# Autodesk Inventor assembly: Assembly1
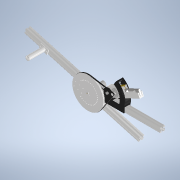
[picture p0: Inventor's stored thumbnail of the model, 180x180]
Saved by Autodesk Inventor 2022 (Build 260153000, 153)
## iProperties
Created: 2022-01-28
Part Number: Assembly1
Document SubType Name: Assembly
Designer: Martijn
Author: Martijn
## Documents named in this file (23)
- D:\phd\git\1dofsetup\Assembly1.iam
- D:\phd\git\1dofsetup\30x30x50.ipt
- D:\phd\git\1dofsetup\bearing_mount.ipt
- D:\phd\git\1dofsetup\force_measurement_thingy.ipt
- D:\phd\git\1dofsetup\NEMA 17.ipt
- D:\phd\git\1dofsetup\pololu-universal-aluminum-mounting-hub-for-5mm-shaft-m3-holes.ipt
- D:\phd\git\1dofsetup\space_plate.ipt
- D:\phd\git\1dofsetup\pololu-universal-aluminum-mounting-hub-for-8mm-shaft-m3-holes.ipt
- D:\phd\git\1dofsetup\SKF_608-2ZZ.ipt
- D:\phd\git\1dofsetup\just_pulley.ipt
- D:\phd\git\1dofsetup\GT2_16T.ipt
- D:\phd\git\1dofsetup\force_measurement_plate.ipt
- D:\phd\git\1dofsetup\load_cell.ipt
- D:\phd\git\1dofsetup\fixation_circle.ipt
- D:\phd\git\1dofsetup\fixation_plate2.ipt
- D:\phd\git\1dofsetup\8mm_to 6.35mm_kaplin.ipt
- D:\phd\git\1dofsetup\axis1.ipt
- D:\phd\git\1dofsetup\Lock Collar 8mm.ipt
- D:\phd\git\1dofsetup\belt.ipt
- D:\phd\git\1dofsetup\handle.ipt
- D:\phd\git\1dofsetup\bearing_mount3.ipt
- D:\phd\git\1dofsetup\axis2.ipt
- D:\phd\git\1dofsetup\load_cell_mounting_block2.ipt
## Components (27 placed, 22 different names)
1. 30x30x50:1 — Mate:96, Flush:34, Mate:106, Flush:35, Flush:36, Mate:118, Flush:38, Mate:131, Flush:44, Mate:132, Mate:133
2. 30x30x50:2 — Mate:29, Flush:10, Mate:107, Mate:108, Flush:37, Flush:39, Mate:120, Flush:40
3. force_measurement_thingy:1 — Mate:99, Mate:100, Mate:101, Mate:102, Mate:103, Mate:104, Mate:135, Angle:1
4. NEMA 17:1 — Mate:6, Mate:102, Mate:103, Mate:104, Mate:105, Mate:112
5. pololu-universal-aluminum-mounting-hub-for-5mm-shaft-m3-holes:1 — Mate:6, Mate:35, Mate:37
6. space_plate:1 — Flush:39, Mate:120, Flush:40, Mate:124, Flush:41, Flush:42
7. pololu-universal-aluminum-mounting-hub-for-8mm-shaft-m3-holes:1 — Mate:115, Mate:116, Mate:117, Mate:123, Flush:43
8. SKF_608-2ZZ:2 — Mate:136
9. just_pulley:1 — Mate:106, Flush:35, Mate:109, Mate:110, Mate:111, Mate:113, Mate:115, Mate:116, Mate:117, Flush:36, Mate:127, Mate:128, Mate:130
10. SKF_608-2ZZ:4 — Mate:110, Mate:127
11. GT2_16T:1 — Mate:36, Mate:105, Mate:114
12. force_measurement_plate:2 — Mate:29, Flush:10, Mate:78, Mate:100, Mate:134, Mate:137, Mate:138
13. load_cell:1 — Mate:101, Mate:135, Angle:1, Mate:139
14. fixation_circle:1 — Mate:35, Mate:36, Mate:37
15. fixation_plate2:1 — Mate:118, Flush:38, Mate:122, Mate:125, Mate:126, Mate:133
16. 8mm_to 6.35mm_kaplin:1 — Mate:122, Mate:129
17. bearing_mount:1 — Mate:107, Mate:108, Mate:109, Mate:111, Flush:37
18. axis1:1 — Mate:75, Mate:77, Flush:30, Mate:99, Mate:136
19. Lock Collar 8mm:1 — Mate:75
20. Lock Collar 8mm:2 — Mate:77, Mate:78, Flush:30, Mate:134
21. belt:1 — Mate:112, Mate:113, Mate:114, Mate:130
22. handle:1 — Mate:96, Flush:34, Mate:123
23. bearing_mount3:1 — Mate:124, Flush:41, Flush:42, Mate:129
24. SKF_608-2ZZ:5 — Mate:125, Mate:126
25. axis2:1 — Mate:128, Flush:43, Mate:140
26. 30x30x50:3 — Mate:131, Flush:44, Mate:132
27. load_cell_mounting_block2:1 — Mate:137, Mate:138, Mate:139
## Relationships (63: Mate 49, Flush 13, Angle 1)
- Mate:6 (1 mm): NEMA 17:1 ↔ pololu-universal-aluminum-mounting-hub-for-5mm-shaft-m3-holes:1
- Mate:29: 30x30x50:2 ↔ force_measurement_plate:2
- Flush:10: 30x30x50:2 ↔ force_measurement_plate:2
- Mate:35: pololu-universal-aluminum-mounting-hub-for-5mm-shaft-m3-holes:1 ↔ fixation_circle:1
- Mate:36: GT2_16T:1 ↔ fixation_circle:1
- Mate:37: pololu-universal-aluminum-mounting-hub-for-5mm-shaft-m3-holes:1 ↔ fixation_circle:1
- Mate:75: axis1:1 ↔ Lock Collar 8mm:1
- Mate:77: axis1:1 ↔ Lock Collar 8mm:2
- Mate:78: force_measurement_plate:2 ↔ Lock Collar 8mm:2
- Flush:30 (0.5 mm): axis1:1 ↔ Lock Collar 8mm:2
- Mate:96: 30x30x50:1 ↔ handle:1
- Flush:34: 30x30x50:1 ↔ handle:1
- Mate:99: force_measurement_thingy:1 ↔ axis1:1
- Mate:100 (0.5 mm): force_measurement_thingy:1 ↔ force_measurement_plate:2
- Mate:101: force_measurement_thingy:1 ↔ load_cell:1
- Mate:102: force_measurement_thingy:1 ↔ NEMA 17:1
- Mate:103: force_measurement_thingy:1 ↔ NEMA 17:1
- Mate:104: force_measurement_thingy:1 ↔ NEMA 17:1
- Mate:105: NEMA 17:1 ↔ GT2_16T:1
- Mate:106: 30x30x50:1 ↔ just_pulley:1
- Flush:35: 30x30x50:1 ↔ just_pulley:1
- Mate:107: 30x30x50:2 ↔ bearing_mount:1
- Mate:108 (-50 mm): 30x30x50:2 ↔ bearing_mount:1
- Mate:109: just_pulley:1 ↔ bearing_mount:1
- Mate:110: just_pulley:1 ↔ SKF_608-2ZZ:4
- Mate:111: just_pulley:1 ↔ bearing_mount:1
- Mate:112: NEMA 17:1 ↔ belt:1
- Mate:113: just_pulley:1 ↔ belt:1
- Mate:114 (0.5 mm): GT2_16T:1 ↔ belt:1
- Mate:115: pololu-universal-aluminum-mounting-hub-for-8mm-shaft-m3-holes:1 ↔ just_pulley:1
- Mate:116: pololu-universal-aluminum-mounting-hub-for-8mm-shaft-m3-holes:1 ↔ just_pulley:1
- Mate:117: pololu-universal-aluminum-mounting-hub-for-8mm-shaft-m3-holes:1 ↔ just_pulley:1
- Flush:36: 30x30x50:1 ↔ just_pulley:1
- Flush:37: 30x30x50:2 ↔ bearing_mount:1
- Mate:118: 30x30x50:1 ↔ fixation_plate2:1
- Flush:38: 30x30x50:1 ↔ fixation_plate2:1
- Flush:39: 30x30x50:2 ↔ space_plate:1
- Mate:120: 30x30x50:2 ↔ space_plate:1
- Flush:40: 30x30x50:2 ↔ space_plate:1
- Mate:122: fixation_plate2:1 ↔ 8mm_to 6.35mm_kaplin:1
- Mate:123 (300 mm): pololu-universal-aluminum-mounting-hub-for-8mm-shaft-m3-holes:1 ↔ handle:1
- Mate:124: space_plate:1 ↔ bearing_mount3:1
- Flush:41: space_plate:1 ↔ bearing_mount3:1
- Flush:42: space_plate:1 ↔ bearing_mount3:1
- Mate:125: fixation_plate2:1 ↔ SKF_608-2ZZ:5
- Mate:126: fixation_plate2:1 ↔ SKF_608-2ZZ:5
- Mate:127 (0.5 mm): just_pulley:1 ↔ SKF_608-2ZZ:4
- Mate:128: just_pulley:1 ↔ axis2:1
- Flush:43: pololu-universal-aluminum-mounting-hub-for-8mm-shaft-m3-holes:1 ↔ axis2:1
- Mate:129 (5 mm): 8mm_to 6.35mm_kaplin:1 ↔ bearing_mount3:1
- Mate:130 (0.5 mm): just_pulley:1 ↔ belt:1
- Mate:131: 30x30x50:1 ↔ 30x30x50:3
- Flush:44: 30x30x50:1 ↔ 30x30x50:3
- Mate:132 (-60 mm): 30x30x50:1 ↔ 30x30x50:3
- Mate:133 (-60 mm): 30x30x50:1 ↔ fixation_plate2:1
- Mate:134: force_measurement_plate:2 ↔ Lock Collar 8mm:2
- Mate:135: force_measurement_thingy:1 ↔ load_cell:1
- Mate:136: SKF_608-2ZZ:2 ↔ axis1:1
- Angle:1 (-180 deg): force_measurement_thingy:1 ↔ load_cell:1
- Mate:137: force_measurement_plate:2 ↔ load_cell_mounting_block2:1
- Mate:138: force_measurement_plate:2 ↔ load_cell_mounting_block2:1
- Mate:139: load_cell:1 ↔ load_cell_mounting_block2:1
- Mate:140: axis2:1
